# Autodesk Inventor assembly: Montagem_correta
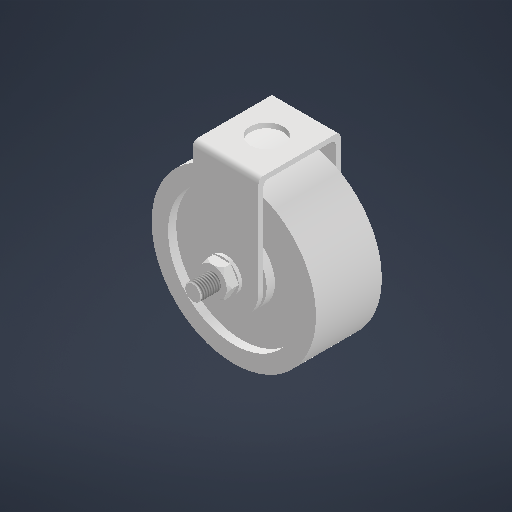
[picture p0: Inventor's stored thumbnail of the model, 512x512]
Saved by Autodesk Inventor 2027.1 (Build 311270010, 270A)
## iProperties
Created: 2026-08-27
Part Number: Montagem_correta
Document SubType Name: Assembly
Designer: labsfiap
Author: labsfiap
## Documents named in this file (7)
- C:\Users\labsfiap\Downloads\Trabalho_1\Montagem_correta.iam
- C:\Users\labsfiap\Downloads\Trabalho_1\6Peça_.ipt
- C:\Users\labsfiap\Downloads\Trabalho_1\5Peça_.ipt
- C:\Users\labsfiap\Downloads\Trabalho_1\4Peça_.ipt
- C:\Users\labsfiap\Downloads\Trabalho_1\3Peça_.ipt
- C:\Users\labsfiap\Downloads\Trabalho_1\2Peça_.ipt
- C:\Users\labsfiap\Downloads\Trabalho_1\1Peça_.ipt
## Components (6 placed, 6 different names)
1. 6Peça_:1 — Coincidente:1, Alinhado:1, Coincidente:2
2. 5Peça_:1 — Coincidente:6, Coincidente:7
3. 4Peça_:1 — Coincidente:4, Coincidente:5, Coincidente:6, Coincidente:8
4. 3Peça_:1 — Coincidente:8, Coincidente:9
5. 2Peça_:1 — Coincidente:2, Coincidente:3, Coincidente:4, Coincidente:5, Coincidente:7, Coincidente:9
6. 1Peça_:1 — Coincidente:1, Alinhado:1, Coincidente:3
## Relationships (10: Mate 9, Flush 1)
- Coincidente:1 [Mate]: 6Peça_:1 ↔ 1Peça_:1
- Alinhado:1 [Flush]: 6Peça_:1 ↔ 1Peça_:1
- Coincidente:2 [Mate]: 6Peça_:1 ↔ 2Peça_:1
- Coincidente:3 [Mate] (2 mm): 2Peça_:1 ↔ 1Peça_:1
- Coincidente:4 [Mate]: 4Peça_:1 ↔ 2Peça_:1
- Coincidente:5 [Mate]: 4Peça_:1 ↔ 2Peça_:1
- Coincidente:6 [Mate]: 5Peça_:1 ↔ 4Peça_:1
- Coincidente:7 [Mate]: 5Peça_:1 ↔ 2Peça_:1
- Coincidente:8 [Mate]: 4Peça_:1 ↔ 3Peça_:1
- Coincidente:9 [Mate]: 3Peça_:1 ↔ 2Peça_:1
